# Autodesk Inventor assembly: MG-Verbindungsstrebe Hinten
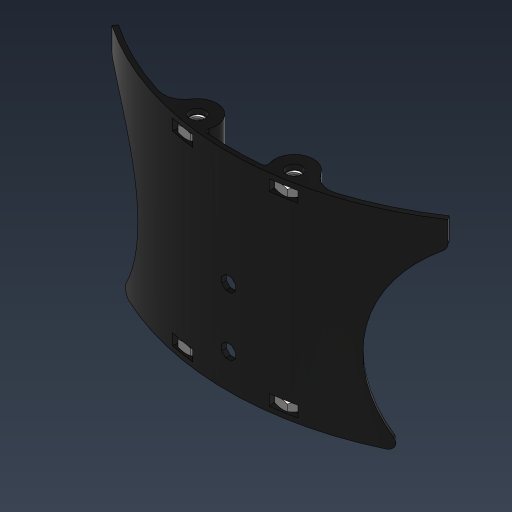
[picture p0: Inventor's stored thumbnail of the model, 512x512]
Saved by Autodesk Inventor 2023.1 (Build 271208000, 208)
## iProperties
Part Number: MG-Verbindungsstrebe Hinten
Material: Generisch
Document SubType Name: Assembly
Designer: rYan
Author: rYan
## Documents named in this file (3)
- D:\TIGERsGIT\mechanics-releases\v2024\Inventor\Robot\Electronics\MG-Verbindungsstrebe Hinten.iam
- D:\TIGERsGIT\mechanics-releases\v2024\Inventor\Robot\Electronics\Verbindungsstrebe Hinten.ipt
- D:\TIGERsGIT\mechanics-releases\v2024\Inventor\Inhaltscenter\de-DE\DIN 934\DIN 934 - M4 x 0,7.ipt
## Components (5 placed, 2 different names)
1. Verbindungsstrebe Hinten:1 — Fluchtend:1, Fluchtend:2, Fluchtend:3, Einfügen:1, Einfügen:2, Einfügen:3, Einfügen:4
2. DIN 934 - ersetzt durch DIN EN 24032/28673/28674 M4:1 — Einfügen:4
3. DIN 934 - ersetzt durch DIN EN 24032/28673/28674 M4:2 — Einfügen:3
4. DIN 934 - ersetzt durch DIN EN 24032/28673/28674 M4:3 — Einfügen:2
5. DIN 934 - ersetzt durch DIN EN 24032/28673/28674 M4:4 — Einfügen:1
## Relationships (7: Insert 4, Flush 3)
- Fluchtend:1 [Flush]: Verbindungsstrebe Hinten:1
- Fluchtend:2 [Flush]: Verbindungsstrebe Hinten:1
- Fluchtend:3 [Flush]: Verbindungsstrebe Hinten:1
- Einfügen:1 [Insert]: Verbindungsstrebe Hinten:1 ↔ DIN 934 - ersetzt durch DIN EN 24032/28673/28674 M4:4
- Einfügen:2 [Insert]: Verbindungsstrebe Hinten:1 ↔ DIN 934 - ersetzt durch DIN EN 24032/28673/28674 M4:3
- Einfügen:3 [Insert]: Verbindungsstrebe Hinten:1 ↔ DIN 934 - ersetzt durch DIN EN 24032/28673/28674 M4:2
- Einfügen:4 [Insert]: Verbindungsstrebe Hinten:1 ↔ DIN 934 - ersetzt durch DIN EN 24032/28673/28674 M4:1
